# Autodesk Inventor assembly: FullSide
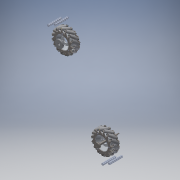
[picture p0: Inventor's stored thumbnail of the model, 180x180]
Saved by Autodesk Inventor 2019 (Build 230136000, 136)
## iProperties
Created: 2019-01-09
Part Number: FullSide
Document SubType Name: Assembly
Designer: james
Author: james
## Documents named in this file (10)
- F:\JimsDesign\2019CHS4089\FullSide.iam
- F:\JimsDesign\Library\AndyMark\am-3922 AM14U4 Inside Plate.ipt
- F:\JimsDesign\Library\AndyMark\am-3921 AM14U4 Outside Plate.ipt
- F:\JimsDesign\Library\AndyMark\3.375in Churro.ipt
- F:\JimsDesign\Library\AndyMark\am-3479L 6 SR Mecanum Left.iam
- F:\JimsDesign\2019CHS4089\OutSpacer.ipt
- F:\JimsDesign\2019CHS4089\InSpace.ipt
- F:\JimsDesign\Library\AndyMark\FR8ZZ Hex Bearing.ipt
- F:\JimsDesign\Library\AndyMark\TB Output Shaft Hex L-Base 2.ipt
- F:\JimsDesign\Library\AndyMark\am-0096a 500 Hex Hub r2.ipt
## Components (14 placed, 9 different names)
1. am-3922 AM14U4 Inside Plate:1 — Mate:9, Mate:10, Mate:11, Mate:16, Mate:19, Mate:20
2. am-3921 AM14U4 Outside Plate:1 — Mate:1, Mate:2, Mate:3, Mate:4, Mate:5, Mate:6, Mate:7, Mate:8, Mate:12, Mate:13, Mate:17, Mate:18, Mate:21, Mate:22
3. 3.375in Churro:1 — Mate:7, Mate:8, Mate:11
4. 3.375in Churro:2 — Mate:1, Mate:2, Mate:9, Mate:10
5. 3.375in Churro:3 — Mate:3, Mate:4
6. 3.375in Churro:4 — Mate:5, Mate:6
7. am-3479L 6 SR Mecanum Left:1 [sub-assembly] — Mate:12, Flush:1, Mate:14, Mate:15
8. am-3479L 6 SR Mecanum Left:2 [sub-assembly] — Flush:1, Mate:13, Mate:24, Mate:25
9. OutSpacer:1 — Mate:14, Mate:15, Mate:16
10. InSpace:1 — Mate:17, Mate:18
11. FR8ZZ Hex Bearing:1 — Mate:19, Mate:20
12. FR8ZZ Hex Bearing:2 — Mate:21, Mate:22, Mate:23, Flush:2
13. TB Output Shaft Hex L-Base 2:1 — Mate:23, Flush:2
14. am-0096a 500 Hex Hub r2:1 — Mate:24, Mate:25
## Relationships (27: Mate 25, Flush 2)
- Mate:1: am-3921 AM14U4 Outside Plate:1 ↔ 3.375in Churro:2
- Mate:2: am-3921 AM14U4 Outside Plate:1 ↔ 3.375in Churro:2
- Mate:3: am-3921 AM14U4 Outside Plate:1 ↔ 3.375in Churro:3
- Mate:4: am-3921 AM14U4 Outside Plate:1 ↔ 3.375in Churro:3
- Mate:5: am-3921 AM14U4 Outside Plate:1 ↔ 3.375in Churro:4
- Mate:6: am-3921 AM14U4 Outside Plate:1 ↔ 3.375in Churro:4
- Mate:7: am-3921 AM14U4 Outside Plate:1 ↔ 3.375in Churro:1
- Mate:8: am-3921 AM14U4 Outside Plate:1 ↔ 3.375in Churro:1
- Mate:9: am-3922 AM14U4 Inside Plate:1 ↔ 3.375in Churro:2
- Mate:10: am-3922 AM14U4 Inside Plate:1 ↔ 3.375in Churro:2
- Mate:11: am-3922 AM14U4 Inside Plate:1 ↔ 3.375in Churro:1
- Mate:12: am-3921 AM14U4 Outside Plate:1 ↔ am-3479L 6 SR Mecanum Left:1
- Flush:1: am-3479L 6 SR Mecanum Left:1 ↔ am-3479L 6 SR Mecanum Left:2
- Mate:13: am-3921 AM14U4 Outside Plate:1 ↔ am-3479L 6 SR Mecanum Left:2
- Mate:14: am-3479L 6 SR Mecanum Left:1 ↔ OutSpacer:1
- Mate:15: am-3479L 6 SR Mecanum Left:1 ↔ OutSpacer:1
- Mate:16: am-3922 AM14U4 Inside Plate:1 ↔ OutSpacer:1
- Mate:17: am-3921 AM14U4 Outside Plate:1 ↔ InSpace:1
- Mate:18: am-3921 AM14U4 Outside Plate:1 ↔ InSpace:1
- Mate:19: am-3922 AM14U4 Inside Plate:1 ↔ FR8ZZ Hex Bearing:1
- Mate:20: am-3922 AM14U4 Inside Plate:1 ↔ FR8ZZ Hex Bearing:1
- Mate:21: am-3921 AM14U4 Outside Plate:1 ↔ FR8ZZ Hex Bearing:2
- Mate:22: am-3921 AM14U4 Outside Plate:1 ↔ FR8ZZ Hex Bearing:2
- Mate:23: FR8ZZ Hex Bearing:2 ↔ TB Output Shaft Hex L-Base 2:1
- Flush:2: FR8ZZ Hex Bearing:2 ↔ TB Output Shaft Hex L-Base 2:1
- Mate:24: am-3479L 6 SR Mecanum Left:2 ↔ am-0096a 500 Hex Hub r2:1
- Mate:25: am-3479L 6 SR Mecanum Left:2 ↔ am-0096a 500 Hex Hub r2:1
